# Autodesk Inventor assembly: DeckelParabol
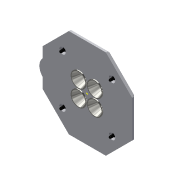
[picture p0: Inventor's stored thumbnail of the model, 180x180]
Saved by Autodesk Inventor 2018.2 (Build 222227000, 227)
## iProperties
Company: Fraunhofer ILT
Created: 2018-10-30
Part Number: DeckelParabol
Material: geeigneten Werkstoff auswählen !
Document SubType Name: Assembly
Designer: N.Grubert
Title: =Description
Author: N.Grubert
## Documents named in this file (4)
- C:\Users\GRUBERT\Documents\COSIMA-Laserstar\CAD\DeckelParabol.iam
- C:\Users\GRUBERT\Documents\COSIMA-Laserstar\CAD\Oktagon_Deckel.ipt
- C:\Users\GRUBERT\Documents\COSIMA-Laserstar\CAD\Parabol.ipt
- C:\Users\GRUBERT\Documents\COSIMA-Laserstar\CAD\Photodiodendummie.ipt
## Components (9 placed, 3 different names)
1. Oktagon_Deckel:1 — Fluchtend:1, Fluchtend:2, Passend:1, Passend:2, Passend:3, Passend:4, Passend:5, Passend:6, Passend:7, Passend:8, Passend:9, Passend:10, Fluchtend:3, Fluchtend:4, Fluchtend:5, Fluchtend:6, Passend:11, Passend:12, Passend:13
2. Parabol:1 — Passend:5, Passend:6
3. Parabol:2 — Passend:4, Passend:7
4. Parabol:3 — Passend:2, Passend:8
5. Parabol:4 — Passend:3, Passend:9
6. Photodiodendummie:1 — Passend:10, Fluchtend:3
7. Photodiodendummie:2 — Fluchtend:6, Passend:12
8. Photodiodendummie:3 — Fluchtend:5, Passend:13
9. Photodiodendummie:4 — Fluchtend:4, Passend:11
## Relationships (19: Mate 13, Flush 6)
- Fluchtend:1 [Flush]: Oktagon_Deckel:1
- Fluchtend:2 [Flush]: Oktagon_Deckel:1
- Passend:1 [Mate]: Oktagon_Deckel:1
- Passend:2 [Mate]: Oktagon_Deckel:1 ↔ Parabol:3
- Passend:3 [Mate]: Oktagon_Deckel:1 ↔ Parabol:4
- Passend:4 [Mate]: Oktagon_Deckel:1 ↔ Parabol:2
- Passend:5 [Mate]: Oktagon_Deckel:1 ↔ Parabol:1
- Passend:6 [Mate]: Oktagon_Deckel:1 ↔ Parabol:1
- Passend:7 [Mate]: Oktagon_Deckel:1 ↔ Parabol:2
- Passend:8 [Mate]: Oktagon_Deckel:1 ↔ Parabol:3
- Passend:9 [Mate]: Oktagon_Deckel:1 ↔ Parabol:4
- Passend:10 [Mate]: Oktagon_Deckel:1 ↔ Photodiodendummie:1
- Fluchtend:3 [Flush]: Oktagon_Deckel:1 ↔ Photodiodendummie:1
- Fluchtend:4 [Flush]: Oktagon_Deckel:1 ↔ Photodiodendummie:4
- Fluchtend:5 [Flush]: Oktagon_Deckel:1 ↔ Photodiodendummie:3
- Fluchtend:6 [Flush]: Oktagon_Deckel:1 ↔ Photodiodendummie:2
- Passend:11 [Mate]: Oktagon_Deckel:1 ↔ Photodiodendummie:4
- Passend:12 [Mate]: Oktagon_Deckel:1 ↔ Photodiodendummie:2
- Passend:13 [Mate]: Oktagon_Deckel:1 ↔ Photodiodendummie:3
